# Autodesk Inventor assembly: totaal auto
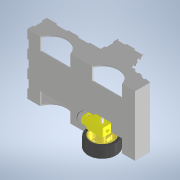
[picture p0: Inventor's stored thumbnail of the model, 180x180]
Saved by Autodesk Inventor 2021 (Build 250183000, 183)
## iProperties
Created: 2022-02-01
Part Number: totaal auto
Document SubType Name: Assembly
Designer: ryan
Author: ryan
## Documents named in this file (6)
- C:\Users\ryan\Desktop\git\projecten\school-P2-auto\modellen\inventor\auto moddellen nieuwste\totaal auto.iam
- C:\Users\ryan\Desktop\git\projecten\school-P2-auto\modellen\inventor\auto moddellen nieuwste\onderkant.ipt
- C:\Users\ryan\Desktop\git\projecten\school-P2-auto\modellen\inventor\auto moddellen nieuwste\zijplaat.ipt
- C:\Users\ryan\Desktop\git\projecten\school-P2-auto\modellen\inventor\geared-dc-motor-for-arduino-applications-1.snapshot.2\Hobi - Motor DC 1.ipt
- C:\Users\ryan\Desktop\git\projecten\school-P2-auto\modellen\inventor\wheel-arduino-1.snapshot.2\Wheel ALL.ipt
- C:\Users\ryan\Desktop\git\projecten\school-P2-auto\modellen\inventor\auto moddellen nieuwste\voorkant.ipt
## Components (6 placed, 5 different names)
1. onderkant:1 — Flush:1, Mate:1, Flush:2, Flush:3, Mate:3, Flush:4, Flush:5, Flush:6, Flush:7, Mate:4
2. zijplaat:1 — Flush:1, Mate:3, Flush:4, Flush:5, Flush:8
3. Hobi - Motor DC 1:1 — Mate:1, Flush:2, Mate:2
4. Wheel ALL:1 — Mate:2
5. voorkant:1 — Flush:3, Flush:6, Flush:7, Flush:8, Flush:9, Flush:10
6. zijplaat:2 — Flush:9, Flush:10, Mate:4
## Relationships (14: Flush 10, Mate 4)
- Flush:1: onderkant:1 ↔ zijplaat:1
- Mate:1: onderkant:1 ↔ Hobi - Motor DC 1:1
- Flush:2: onderkant:1 ↔ Hobi - Motor DC 1:1
- Mate:2: Hobi - Motor DC 1:1 ↔ Wheel ALL:1
- Flush:3: onderkant:1 ↔ voorkant:1
- Mate:3: onderkant:1 ↔ zijplaat:1
- Flush:4: onderkant:1 ↔ zijplaat:1
- Flush:5: onderkant:1 ↔ zijplaat:1
- Flush:6: onderkant:1 ↔ voorkant:1
- Flush:7: onderkant:1 ↔ voorkant:1
- Flush:8: zijplaat:1 ↔ voorkant:1
- Flush:9: voorkant:1 ↔ zijplaat:2
- Flush:10: voorkant:1 ↔ zijplaat:2
- Mate:4: onderkant:1 ↔ zijplaat:2
